# Autodesk Inventor assembly: DT Assembly
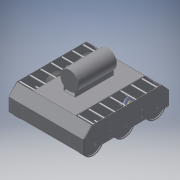
[picture p0: Inventor's stored thumbnail of the model, 180x180]
Saved by Autodesk Inventor 2016 (Build 200138000, 138)
## iProperties
Created: 2018-05-05
Part Number: DT Assembly
Document SubType Name: Assembly
Designer: Kade
Author: Kade
## Documents named in this file (11)
- F:\Robotics\Off Season\Blannon\DT Assembly.iam
- F:\Robotics\Off Season\Blannon\DT Side Assembly.iam
- F:\Robotics\Off Season\Blannon\End Plates.ipt
- F:\Robotics\Off Season\Blannon\DT Side Assembly_MIR1.iam
- F:\Robotics\Off Season\Blannon\BellyPan Lexan.ipt
- F:\Robotics\Off Season\Blannon\Side Gurad.ipt
- F:\Robotics\Off Season\Blannon\Deep Cycle Battery.ipt
- F:\Robotics\Off Season\Blannon\FRC Battery.ipt
- F:\Robotics\Off Season\Blannon\compressor.ipt
- F:\Robotics\Off Season\Blannon\air tank mount.ipt
- F:\Robotics\Off Season\Blannon\Tank.ipt
## Components (13 placed, 10 different names)
1. DT Side Assembly:1 [sub-assembly] — Mate:1, Flush:14, Mate:3, Flush:15, Mate:5, Mate:6, Flush:20, Mate:9, Mate:24, Flush:25, Mate:27, Flush:27
2. End Plates:1 — Mate:1, Flush:14, Mate:5, Insert:1, Flush:18, Flush:19, Flush:21, Mate:7, Flush:24, Mate:22
3. End Plates:2 — Mate:3, Flush:15, Mate:6, Flush:16, Mate:8, Mate:26
4. DT Side Assembly_MIR1:1 [sub-assembly] — Insert:1, Flush:18, Flush:22, Flush:23, Mate:23, Mate:28
5. BellyPan Lexan:1 — Flush:19, Flush:20, Flush:21, Mate:10, Mate:18, Mate:21
6. Side Gurad:1 — Flush:23, Angle:2, Mate:7, Mate:29
7. Side Gurad:2 — Flush:22, Angle:1, Mate:8
8. FRC Battery:1 — Mate:10, Flush:25, Flush:26
9. compressor:1 — Flush:26, Mate:26, Mate:27
10. compressor:2 — Mate:18, Mate:24, Mate:25
11. Tank:1 — Flush:28, Flush:29, Mate:30
12. Deep Cycle Battery:2 — Mate:21, Mate:22, Mate:23, Mate:25
13. air tank mount:1 — Flush:27, Mate:28, Mate:29, Flush:28, Flush:29, Mate:30
## Relationships (37: Mate 19, Flush 15, Angle 2, Insert 1)
- Mate:1: DT Side Assembly:1 ↔ End Plates:1
- Flush:14: DT Side Assembly:1 ↔ End Plates:1
- Mate:3: DT Side Assembly:1 ↔ End Plates:2
- Flush:15: DT Side Assembly:1 ↔ End Plates:2
- Mate:5 (-25.4 mm): DT Side Assembly:1 ↔ End Plates:1
- Mate:6 (-25.4 mm): DT Side Assembly:1 ↔ End Plates:2
- Flush:16 (355.6 mm): End Plates:2
- Insert:1: End Plates:1 ↔ DT Side Assembly_MIR1:1
- Flush:18: End Plates:1 ↔ DT Side Assembly_MIR1:1
- Flush:19 (-3.175 mm): End Plates:1 ↔ BellyPan Lexan:1
- Flush:20 (-3.175 mm): DT Side Assembly:1 ↔ BellyPan Lexan:1
- Flush:21: End Plates:1 ↔ BellyPan Lexan:1
- Flush:22 (3.175 mm): DT Side Assembly_MIR1:1 ↔ Side Gurad:2
- Flush:23 (3.175 mm): DT Side Assembly_MIR1:1 ↔ Side Gurad:1
- Angle:1 (137 deg): Side Gurad:2
- Angle:2 (45 deg): Side Gurad:1
- Mate:7: End Plates:1 ↔ Side Gurad:1
- Mate:8: End Plates:2 ↔ Side Gurad:2
- Mate:9: DT Side Assembly:1
- Flush:24: End Plates:1
- Mate:10: BellyPan Lexan:1 ↔ FRC Battery:1
- Mate:18: BellyPan Lexan:1 ↔ compressor:2
- Mate:21: BellyPan Lexan:1 ↔ Deep Cycle Battery:2
- Mate:22 (50.8 mm): End Plates:1 ↔ Deep Cycle Battery:2
- Mate:23 (6.35 mm): DT Side Assembly_MIR1:1 ↔ Deep Cycle Battery:2
- Mate:24 (50.8 mm): DT Side Assembly:1 ↔ compressor:2
- Mate:25 (50.8 mm): compressor:2 ↔ Deep Cycle Battery:2
- Flush:25 (-127 mm): DT Side Assembly:1 ↔ FRC Battery:1
- Flush:26 (203.2 mm): FRC Battery:1 ↔ compressor:1
- Mate:26 (50.8 mm): End Plates:2 ↔ compressor:1
- Mate:27 (50.8 mm): DT Side Assembly:1 ↔ compressor:1
- Flush:27: DT Side Assembly:1 ↔ air tank mount:1
- Mate:28: DT Side Assembly_MIR1:1 ↔ air tank mount:1
- Mate:29: Side Gurad:1 ↔ air tank mount:1
- Flush:28 (146.05 mm): Tank:1 ↔ air tank mount:1
- Flush:29 (147.32 mm): Tank:1 ↔ air tank mount:1
- Mate:30: Tank:1 ↔ air tank mount:1
